# Autodesk Inventor assembly: DriverStation-ver1-1111-2021
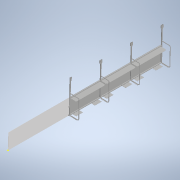
[picture p0: Inventor's stored thumbnail of the model, 180x180]
Saved by Autodesk Inventor 2021 (Build 250183000, 183)
## iProperties
Created: 2021-02-25
Part Number: DriverStation-ver1-1111-2021
Document SubType Name: Assembly
Designer: CMurray
Author: CMurray
## Documents named in this file (6)
- F:\PHRC CADD 2021\2021 Game Design Challenge\Player Station\Assemblies\DriverStation-ver1-1111-2021.iam
- F:\PHRC CADD 2021\2021 Game Design Challenge\Player Station\Parts\PSBase-ver1-1111-2021.iam
- F:\PHRC CADD 2021\2021 Game Design Challenge\Player Station\Parts\PSBaseArmLeft-ver1-1111-2021.iam
- F:\PHRC CADD 2021\2021 Game Design Challenge\Player Station\Parts\PSBaseArmRight-ver1-1111-2021.iam
- F:\PHRC CADD 2021\2021 Game Design Challenge\Player Station\Parts\PSHalfWall-ver1-1111-2021.ipt
- PSBase-ver1-1111-2021.ipt
## Components (8 placed, 4 different names)
1. PSBase-ver1-1111-2021:1 [sub-assembly] — Flush:1, Mate:1, Mate:2, Flush:2, Mate:3, Mate:4, Flush:3, Flush:7, Flush:8
2. PSBaseArmLeft-ver1-1111-2021:1 [sub-assembly] — Flush:1, Mate:1, Mate:2, Mate:14
3. PSBaseArmRight-ver1-1111-2021:1 [sub-assembly] — Flush:2, Mate:3, Mate:4, Mate:5, Mate:6
4. PSBase-ver1-1111-2021:2 [sub-assembly] — Flush:3, Mate:5, Mate:6, Flush:4, Mate:7, Mate:8, Flush:5
5. PSBaseArmRight-ver1-1111-2021:2 [sub-assembly] — Flush:4, Mate:7, Mate:8, Mate:9, Mate:10
6. PSBase-ver1-1111-2021:3 [sub-assembly] — Flush:5, Mate:9, Mate:10, Flush:6, Mate:11, Mate:12
7. PSBaseArmRight-ver1-1111-2021:3 [sub-assembly] — Flush:6, Mate:11, Mate:12, Mate:13, Angle:1
8. PSHalfWall-ver1-1111-2021:1 — Flush:7, Flush:8, Mate:14
## Relationships (23: Mate 14, Flush 8, Angle 1)
- Flush:1: PSBase-ver1-1111-2021:1 ↔ PSBaseArmLeft-ver1-1111-2021:1
- Mate:1: PSBase-ver1-1111-2021:1 ↔ PSBaseArmLeft-ver1-1111-2021:1
- Mate:2: PSBase-ver1-1111-2021:1 ↔ PSBaseArmLeft-ver1-1111-2021:1
- Flush:2: PSBase-ver1-1111-2021:1 ↔ PSBaseArmRight-ver1-1111-2021:1
- Mate:3: PSBase-ver1-1111-2021:1 ↔ PSBaseArmRight-ver1-1111-2021:1
- Mate:4: PSBase-ver1-1111-2021:1 ↔ PSBaseArmRight-ver1-1111-2021:1
- Flush:3: PSBase-ver1-1111-2021:1 ↔ PSBase-ver1-1111-2021:2
- Mate:5: PSBaseArmRight-ver1-1111-2021:1 ↔ PSBase-ver1-1111-2021:2
- Mate:6: PSBaseArmRight-ver1-1111-2021:1 ↔ PSBase-ver1-1111-2021:2
- Flush:4: PSBase-ver1-1111-2021:2 ↔ PSBaseArmRight-ver1-1111-2021:2
- Mate:7: PSBase-ver1-1111-2021:2 ↔ PSBaseArmRight-ver1-1111-2021:2
- Mate:8: PSBase-ver1-1111-2021:2 ↔ PSBaseArmRight-ver1-1111-2021:2
- Flush:5: PSBase-ver1-1111-2021:2 ↔ PSBase-ver1-1111-2021:3
- Mate:9: PSBaseArmRight-ver1-1111-2021:2 ↔ PSBase-ver1-1111-2021:3
- Mate:10: PSBaseArmRight-ver1-1111-2021:2 ↔ PSBase-ver1-1111-2021:3
- Flush:6: PSBase-ver1-1111-2021:3 ↔ PSBaseArmRight-ver1-1111-2021:3
- Mate:11: PSBase-ver1-1111-2021:3 ↔ PSBaseArmRight-ver1-1111-2021:3
- Mate:12: PSBase-ver1-1111-2021:3 ↔ PSBaseArmRight-ver1-1111-2021:3
- Mate:13: PSBaseArmRight-ver1-1111-2021:3
- Angle:1 (0 deg): PSBaseArmRight-ver1-1111-2021:3
- Flush:7: PSBase-ver1-1111-2021:1 ↔ PSHalfWall-ver1-1111-2021:1
- Flush:8: PSBase-ver1-1111-2021:1 ↔ PSHalfWall-ver1-1111-2021:1
- Mate:14: PSBaseArmLeft-ver1-1111-2021:1 ↔ PSHalfWall-ver1-1111-2021:1
